# Autodesk Inventor assembly: MK8 Red Extruder Bowden
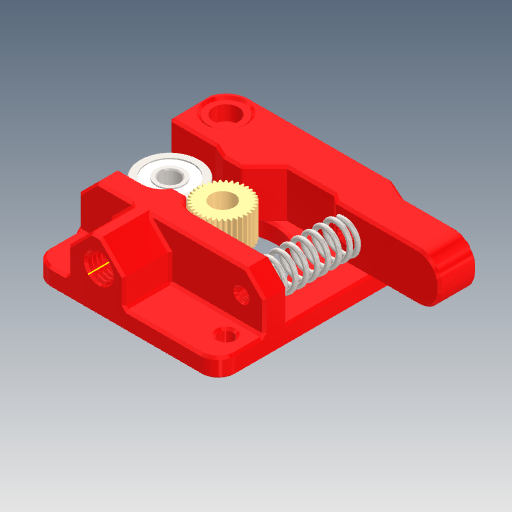
[picture p0: Inventor's stored thumbnail of the model, 512x512]
Saved by Autodesk Inventor 2021 (Build 250183000, 183)
## iProperties
Created: 2021-04-09
Part Number: MK8 Red Extruder Bowden
Document SubType Name: Assembly
Designer: WubbGmbaa
Sending System: SolidWorks 2018
Last Author: daves
Last Saved: 2021-04-09
Author: WubbGmbaa
## Documents named in this file (7)
- G:\Misc\makerspace\TAZ\hybrid-hotend-refactor\ref\MK8 Red Extruder Bowden.iam
- G:\Misc\makerspace\TAZ\hybrid-hotend-refactor\ref\extruder\Extrusor - P1 -MK8^MK8 Red Extruder Bowden.ipt
- G:\Misc\makerspace\TAZ\hybrid-hotend-refactor\ref\extruder\Extrusor - P2 -MK8^MK8 Red Extruder Bowden.ipt
- G:\Misc\makerspace\TAZ\hybrid-hotend-refactor\ref\extruder\Extrusor - P3 -MK8^MK8 Red Extruder Bowden.ipt
- G:\Misc\makerspace\TAZ\hybrid-hotend-refactor\ref\extruder\Toothed Filament Feed^MK8 Red Extruder Bowden.ipt
- G:\Misc\makerspace\TAZ\hybrid-hotend-refactor\ref\extruder\U604zz^MK8 Red Extruder Bowden.ipt
- G:\Misc\makerspace\TAZ\hybrid-hotend-refactor\ref\extruder\Mola^MK8 Red Extruder Bowden.ipt
## Components (6 placed, 6 different names)
1. Extrusor - P1 -MK8^MK8 Red Extruder Bowden:2 — Mate:1
2. Extrusor - P2 -MK8^MK8 Red Extruder Bowden:1
3. Extrusor - P3 -MK8^MK8 Red Extruder Bowden:1
4. Toothed Filament Feed^MK8 Red Extruder Bowden:1
5. U604zz^MK8 Red Extruder Bowden:1
6. Mola^MK8 Red Extruder Bowden:1
## Relationships (1: Mate 1)
- Mate:1: Extrusor - P1 -MK8^MK8 Red Extruder Bowden:2
